# Autodesk Inventor assembly: manipulator
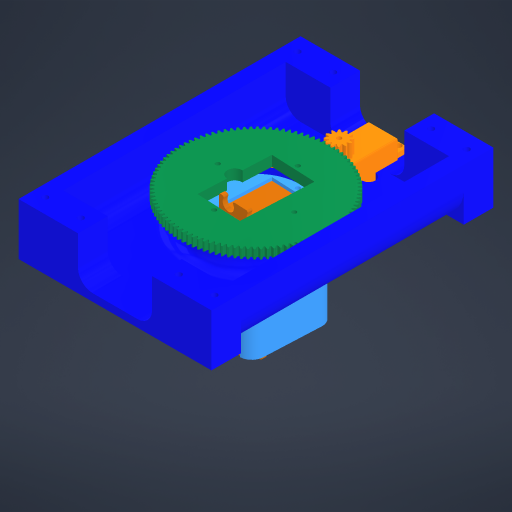
[picture p0: Inventor's stored thumbnail of the model, 512x512]
Saved by Autodesk Inventor 2024 (Build 280153000, 153)
## iProperties
Created: 2023-11-07
Part Number: manipulator
Document SubType Name: Assembly
Designer: user
Author: user
## Documents named in this file (8)
- D:\Docs\Robot\3d_v2\machine_body\manipulator.iam
- D:\Docs\Robot\3d_v2\machine_body\manipulator\platform.ipt
- D:\Docs\Robot\3d_v2\machine_body\manipulator\ring.ipt
- D:\Docs\Robot\3d_v2\machine_body\manipulator\driven_gear.ipt
- D:\Docs\Robot\3d_v2\default_components\servo_80kg.ipt
- D:\Docs\Robot\3d_v2\machine_body\manipulator\bushing_asm.iam
- D:\Docs\Robot\3d_v2\default_components\servo_40kg.ipt
- D:\Docs\Robot\3d_v2\machine_body\manipulator\driving_gear.ipt
## Components (8 placed, 7 different names)
1. platform:2 — Совмещение:1, Совмещение:2, Совмещение:3, Заподлицо:1, Заподлицо:2, Совмещение:4, Вставка:2, Вставка:4, Вставка:5
2. ring:1 — Заподлицо:1, Заподлицо:2, Вставка:1
3. driven_gear:1 — Вставка:1, Совмещение:5, Совмещение:6
4. ring:2 — Совмещение:4, Вставка:2, Вставка:3
5. servo_80kg:1 — Совмещение:5, Совмещение:6, Совмещение:7, Заподлицо:3
6. bushing_asm:1 [sub-assembly] — Вставка:3, Совмещение:7, Заподлицо:3
7. servo_40kg:1 — Вставка:4, Вставка:5, Вставка:6
8. driving_gear:1 — Вставка:6
## Relationships (16: Mate 7, Insert 6, Flush 3)
- Совмещение:1 [Mate]: platform:2
- Совмещение:2 [Mate]: platform:2
- Совмещение:3 [Mate]: platform:2
- Заподлицо:1 [Flush]: platform:2 ↔ ring:1
- Заподлицо:2 [Flush]: platform:2 ↔ ring:1
- Вставка:1 [Insert]: ring:1 ↔ driven_gear:1
- Совмещение:4 [Mate]: platform:2 ↔ ring:2
- Вставка:2 [Insert]: platform:2 ↔ ring:2
- Совмещение:5 [Mate]: driven_gear:1 ↔ servo_80kg:1
- Совмещение:6 [Mate]: driven_gear:1 ↔ servo_80kg:1
- Вставка:3 [Insert]: ring:2 ↔ bushing_asm:1
- Совмещение:7 [Mate]: servo_80kg:1 ↔ bushing_asm:1
- Заподлицо:3 [Flush]: servo_80kg:1 ↔ bushing_asm:1
- Вставка:4 [Insert]: platform:2 ↔ servo_40kg:1
- Вставка:5 [Insert]: platform:2 ↔ servo_40kg:1
- Вставка:6 [Insert]: servo_40kg:1 ↔ driving_gear:1
